# Autodesk Inventor assembly: Chassi 1-14-2020
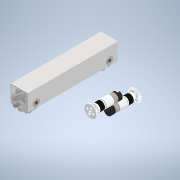
[picture p0: Inventor's stored thumbnail of the model, 180x180]
Saved by Autodesk Inventor 2020.2 (Build 242310000, 310)
## iProperties
Created: 2019-12-09
Part Number: Chassi 1-14-2020
Document SubType Name: Assembly
Designer: deli
Author: deli
## Documents named in this file (14)
- C:\Users\deli\OneDrive - Eastside Preparatory School\FTC\Chassi\Chassi 1-14-2020.iam
- C:\Users\deli\OneDrive - Eastside Preparatory School\FTC\Chassi\38007_txm-aluminum bevel gearing.ipt
- C:\Users\deli\OneDrive - Eastside Preparatory School\FTC\Chassi\am-3215 6mm D bore Double Nub.ipt
- C:\Users\deli\OneDrive - Eastside Preparatory School\FTC\Chassi\am-3637 NeveRest Orbital 20 Gearmotor REV2.ipt
- C:\Users\deli\OneDrive - Eastside Preparatory School\Documents\Personal\Maslow\Side Channel.ipt
- C:\Users\deli\OneDrive - Eastside Preparatory School\FTC\Chassi\100 mm mecanum wheel.ipt
- C:\Users\deli\OneDrive - Eastside Preparatory School\FTC\Chassi\0_500_Hex_ID_x_1_125_OD_x_0_313_WD_Flanged_Bearing_v2_217-3875 v1.ipt
- C:\Users\deli\OneDrive - Eastside Preparatory School\FTC\Chassi\MecanumSideplates v1.ipt
- C:\Users\deli\OneDrive - Eastside Preparatory School\FTC\Chassi\MecanumSideplates with 18t belt gear.ipt
- C:\Users\deli\OneDrive - Eastside Preparatory School\FTC\Chassi\Axel for wheels 1_2_Hex_x_0_201_ID_ThunderHex_Stock_36_217-4017.ipt
- C:\Users\deli\OneDrive - Eastside Preparatory School\FTC\Chassi\100 mm mecanum wheel_MIR.ipt
- C:\Users\deli\OneDrive - Eastside Preparatory School\FTC\Chassi\38007_txm-aluminum bevel gearing_MIR.ipt
- C:\Users\deli\OneDrive - Eastside Preparatory School\FTC\Chassi\am-3215 6mm D bore Double Nub_MIR.ipt
- C:\Users\deli\OneDrive - Eastside Preparatory School\FTC\Chassi\am-3637 NeveRest Orbital 20 Gearmotor REV2_MIR.ipt
## Components (19 placed, 13 different names)
1. 38007_txm-aluminum bevel gearing:2 — Mate:4, Mate:5
2. am-3215 6mm D bore Double Nub:2 — Mate:1, Mate:2, Mate:3, Mate:4, Mate:5
3. am-3637 NeveRest Orbital 20 Gearmotor REV2:2 — Mate:1, Mate:2, Mate:3
4. Side Channel:1 — Mate:61, Mate:62, Mate:67, Mate:68
5. 0_500_Hex_ID_x_1_125_OD_x_0_313_WD_Flanged_Bearing_v2_217-3875 v1:3 — Flush:5, Mate:67, Mate:68
6. 0_500_Hex_ID_x_1_125_OD_x_0_313_WD_Flanged_Bearing_v2_217-3875 v1:4
7. MecanumSideplates v1:2 — Mate:65
8. MecanumSideplates with 18t belt gear:2 — Mate:64, Mate:66
9. Axel for wheels 1_2_Hex_x_0_201_ID_ThunderHex_Stock_36_217-4017:2 — Mate:63, Flush:5
10. 100 mm mecanum wheel:3
11. 0_500_Hex_ID_x_1_125_OD_x_0_313_WD_Flanged_Bearing_v2_217-3875 v1:5 — Mate:61, Flush:4, Mate:62
12. 0_500_Hex_ID_x_1_125_OD_x_0_313_WD_Flanged_Bearing_v2_217-3875 v1:6
13. MecanumSideplates v1:3
14. MecanumSideplates with 18t belt gear:3
15. Axel for wheels 1_2_Hex_x_0_201_ID_ThunderHex_Stock_36_217-4017:3 — Flush:4
16. 100 mm mecanum wheel_MIR:1 — Mate:63, Mate:64, Mate:65, Mate:66
17. 38007_txm-aluminum bevel gearing_MIR:1 — Mate:69, Mate:70
18. am-3215 6mm D bore Double Nub_MIR:1 — Mate:69, Mate:70, Mate:71, Mate:72, Mate:73
19. am-3637 NeveRest Orbital 20 Gearmotor REV2_MIR:1 — Mate:71, Mate:72, Mate:73
## Relationships (48: Mate 36, Angle 8, Flush 4)
- Mate:1: am-3215 6mm D bore Double Nub:2 ↔ am-3637 NeveRest Orbital 20 Gearmotor REV2:2
- Mate:2: am-3215 6mm D bore Double Nub:2 ↔ am-3637 NeveRest Orbital 20 Gearmotor REV2:2
- Mate:3: am-3215 6mm D bore Double Nub:2 ↔ am-3637 NeveRest Orbital 20 Gearmotor REV2:2
- Mate:4: 38007_txm-aluminum bevel gearing:2 ↔ am-3215 6mm D bore Double Nub:2
- Mate:5: 38007_txm-aluminum bevel gearing:2 ↔ am-3215 6mm D bore Double Nub:2
- [Mate]: 0_500_Hex_ID_x_1_125_OD_x_0_313_WD_Flanged_Bearing_v2_217-3875 v1:4 ↔ MecanumSideplates v1:2
- [Mate]: 0_500_Hex_ID_x_1_125_OD_x_0_313_WD_Flanged_Bearing_v2_217-3875 v1:4 ↔ Axel for wheels 1_2_Hex_x_0_201_ID_ThunderHex_Stock_36_217-4017:2
- [Angle] (0 deg): 0_500_Hex_ID_x_1_125_OD_x_0_313_WD_Flanged_Bearing_v2_217-3875 v1:4 ↔ Axel for wheels 1_2_Hex_x_0_201_ID_ThunderHex_Stock_36_217-4017:2
- [Mate]: MecanumSideplates v1:2 ↔ Axel for wheels 1_2_Hex_x_0_201_ID_ThunderHex_Stock_36_217-4017:2
- [Angle] (0 deg): MecanumSideplates v1:2 ↔ Axel for wheels 1_2_Hex_x_0_201_ID_ThunderHex_Stock_36_217-4017:2
- [Mate]: MecanumSideplates with 18t belt gear:2 ↔ Axel for wheels 1_2_Hex_x_0_201_ID_ThunderHex_Stock_36_217-4017:2
- [Angle] (0 deg): MecanumSideplates with 18t belt gear:2 ↔ Axel for wheels 1_2_Hex_x_0_201_ID_ThunderHex_Stock_36_217-4017:2
- [Mate]: 0_500_Hex_ID_x_1_125_OD_x_0_313_WD_Flanged_Bearing_v2_217-3875 v1:3 ↔ Axel for wheels 1_2_Hex_x_0_201_ID_ThunderHex_Stock_36_217-4017:2
- [Angle] (0 deg): 0_500_Hex_ID_x_1_125_OD_x_0_313_WD_Flanged_Bearing_v2_217-3875 v1:3 ↔ Axel for wheels 1_2_Hex_x_0_201_ID_ThunderHex_Stock_36_217-4017:2
- [Flush]: 0_500_Hex_ID_x_1_125_OD_x_0_313_WD_Flanged_Bearing_v2_217-3875 v1:4 ↔ Axel for wheels 1_2_Hex_x_0_201_ID_ThunderHex_Stock_36_217-4017:2
- [Mate]: 100 mm mecanum wheel:3 ↔ 0_500_Hex_ID_x_1_125_OD_x_0_313_WD_Flanged_Bearing_v2_217-3875 v1:5
- [Mate]: 100 mm mecanum wheel:3 ↔ MecanumSideplates v1:3
- [Mate]: 100 mm mecanum wheel:3 ↔ MecanumSideplates v1:3
- [Mate]: 100 mm mecanum wheel:3 ↔ MecanumSideplates v1:3
- [Mate]: 0_500_Hex_ID_x_1_125_OD_x_0_313_WD_Flanged_Bearing_v2_217-3875 v1:6 ↔ MecanumSideplates v1:3
- [Mate]: 100 mm mecanum wheel:3 ↔ MecanumSideplates with 18t belt gear:3
- [Mate]: 100 mm mecanum wheel:3 ↔ MecanumSideplates with 18t belt gear:3
- [Mate]: 100 mm mecanum wheel:3 ↔ MecanumSideplates with 18t belt gear:3
- [Mate]: 0_500_Hex_ID_x_1_125_OD_x_0_313_WD_Flanged_Bearing_v2_217-3875 v1:6 ↔ Axel for wheels 1_2_Hex_x_0_201_ID_ThunderHex_Stock_36_217-4017:3
- [Angle] (0 deg): 0_500_Hex_ID_x_1_125_OD_x_0_313_WD_Flanged_Bearing_v2_217-3875 v1:6 ↔ Axel for wheels 1_2_Hex_x_0_201_ID_ThunderHex_Stock_36_217-4017:3
- [Mate]: MecanumSideplates v1:3 ↔ Axel for wheels 1_2_Hex_x_0_201_ID_ThunderHex_Stock_36_217-4017:3
- [Angle] (0 deg): MecanumSideplates v1:3 ↔ Axel for wheels 1_2_Hex_x_0_201_ID_ThunderHex_Stock_36_217-4017:3
- [Mate]: 100 mm mecanum wheel:3 ↔ Axel for wheels 1_2_Hex_x_0_201_ID_ThunderHex_Stock_36_217-4017:3
- [Mate]: MecanumSideplates with 18t belt gear:3 ↔ Axel for wheels 1_2_Hex_x_0_201_ID_ThunderHex_Stock_36_217-4017:3
- [Angle] (0 deg): MecanumSideplates with 18t belt gear:3 ↔ Axel for wheels 1_2_Hex_x_0_201_ID_ThunderHex_Stock_36_217-4017:3
- [Mate]: 0_500_Hex_ID_x_1_125_OD_x_0_313_WD_Flanged_Bearing_v2_217-3875 v1:5 ↔ Axel for wheels 1_2_Hex_x_0_201_ID_ThunderHex_Stock_36_217-4017:3
- [Angle] (0 deg): 0_500_Hex_ID_x_1_125_OD_x_0_313_WD_Flanged_Bearing_v2_217-3875 v1:5 ↔ Axel for wheels 1_2_Hex_x_0_201_ID_ThunderHex_Stock_36_217-4017:3
- [Flush]: 0_500_Hex_ID_x_1_125_OD_x_0_313_WD_Flanged_Bearing_v2_217-3875 v1:6 ↔ Axel for wheels 1_2_Hex_x_0_201_ID_ThunderHex_Stock_36_217-4017:3
- Mate:61: Side Channel:1 ↔ 0_500_Hex_ID_x_1_125_OD_x_0_313_WD_Flanged_Bearing_v2_217-3875 v1:5
- Flush:4: 0_500_Hex_ID_x_1_125_OD_x_0_313_WD_Flanged_Bearing_v2_217-3875 v1:5 ↔ Axel for wheels 1_2_Hex_x_0_201_ID_ThunderHex_Stock_36_217-4017:3
- Mate:62: Side Channel:1 ↔ 0_500_Hex_ID_x_1_125_OD_x_0_313_WD_Flanged_Bearing_v2_217-3875 v1:5
- Mate:63: Axel for wheels 1_2_Hex_x_0_201_ID_ThunderHex_Stock_36_217-4017:2 ↔ 100 mm mecanum wheel_MIR:1
- Mate:64: MecanumSideplates with 18t belt gear:2 ↔ 100 mm mecanum wheel_MIR:1
- Mate:65: MecanumSideplates v1:2 ↔ 100 mm mecanum wheel_MIR:1
- Mate:66: MecanumSideplates with 18t belt gear:2 ↔ 100 mm mecanum wheel_MIR:1
- Flush:5: 0_500_Hex_ID_x_1_125_OD_x_0_313_WD_Flanged_Bearing_v2_217-3875 v1:3 ↔ Axel for wheels 1_2_Hex_x_0_201_ID_ThunderHex_Stock_36_217-4017:2
- Mate:67: Side Channel:1 ↔ 0_500_Hex_ID_x_1_125_OD_x_0_313_WD_Flanged_Bearing_v2_217-3875 v1:3
- Mate:68: Side Channel:1 ↔ 0_500_Hex_ID_x_1_125_OD_x_0_313_WD_Flanged_Bearing_v2_217-3875 v1:3
- Mate:69: 38007_txm-aluminum bevel gearing_MIR:1 ↔ am-3215 6mm D bore Double Nub_MIR:1
- Mate:70: 38007_txm-aluminum bevel gearing_MIR:1 ↔ am-3215 6mm D bore Double Nub_MIR:1
- Mate:71: am-3215 6mm D bore Double Nub_MIR:1 ↔ am-3637 NeveRest Orbital 20 Gearmotor REV2_MIR:1
- Mate:72: am-3215 6mm D bore Double Nub_MIR:1 ↔ am-3637 NeveRest Orbital 20 Gearmotor REV2_MIR:1
- Mate:73: am-3215 6mm D bore Double Nub_MIR:1 ↔ am-3637 NeveRest Orbital 20 Gearmotor REV2_MIR:1
## Named parameters: d45_d25 = 0 mm, d49_d30 = 0 mm, d50_d31 = 0 deg, d51_d33 = 0 mm, d52_d34 = 0 deg, d54_d36 = 0 mm, d55_d37 = 0 deg, d56_d38 = 0 mm, d57_d39 = 0 deg, d58_d40 = 0 mm, d59_d7 = 0 mm, d60_d11 = 0 mm, d61_d12 = 0 mm, d62_d13 = 0 mm, d63_d25 = 0 mm, d64_d26 = 0 mm, d65_d28 = 0 mm, d66_d29 = 0 mm, d67_d30 = 0 mm, d68_d31 = 0 deg, d69_d33 = 0 mm, d70_d34 = 0 deg, d71_d35 = 0 mm, d72_d36 = 0 mm, d73_d37 = 0 deg, d74_d38 = 0 mm, d75_d39 = 0 deg, d76_d40 = 0 mm
